# Autodesk Inventor assembly: Curved Assembly
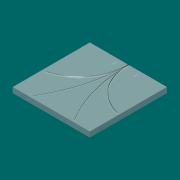
[picture p0: Inventor's stored thumbnail of the model, 180x180]
Saved by Autodesk Inventor 2016 (Build 200138000, 138)
## iProperties
Created: 2015-08-14
Part Number: Curved Assembly
Document SubType Name: Assembly
Designer: Cosmic
Author: Cosmic
## Documents named in this file (4)
- C:\Users\sawaiz\oneDrive\projects\scintillatorPanel\treePanel.iam
- C:\Users\sawaiz\oneDrive\projects\scintillatorPanel\treePanel.ipt
- C:\Users\sawaiz\oneDrive\projects\scintillatorPanel\treeFiberBundle.iam
- C:\Users\sawaiz\oneDrive\projects\scintillatorPanel\Scintillator.xlsx
## Components (2 placed, 2 different names)
1. treePanel:1 — Angle:1, Tangent:2, Flush:1, Mate:27
2. treeFiberBundle:1 [sub-assembly] — Angle:1, Tangent:2, Flush:1, Mate:27
## Relationships (4: Angle 1, Tangent 1, Flush 1, Mate 1)
- Angle:1 (-90 deg): treePanel:1 ↔ treeFiberBundle:1
- Tangent:2 (0.15 mm): treePanel:1 ↔ treeFiberBundle:1
- Flush:1: treePanel:1 ↔ treeFiberBundle:1
- Mate:27: treePanel:1 ↔ treeFiberBundle:1
## Named parameters: OpticalFiberClearence = 0.15 mm, MPPCClearence = 0.075 mm, FiberSensorClerence = 0.5 mm, OpticalFiberDiameter = 1 mm, ScintillatorThickness = 10 mm, SmallTrackDiameter = 175 mm, LargeTrackRatio = 3, ScintillatorEdgeClearence = 3 mm, ScintillatorWidth = 145 mm, ScintillatorHeight = 145 mm, ShallowTrackDepth = 1.3 mm, MPPCSensorClearence = 1.45 mm, MPPCSensorOffsett = 2.105 mm, MPPCWidth = 5.9 mm, MPPCHeight = 6.55 mm, FiberEdgeOffsett = 5 mm, MPPCDepth = 0 mm, LongFiberAngle = 30 deg, ShortFiberAngle = 78 deg, LoopLargeTrackRatio = 1.1, LoopSmallTrackDiameter = 90 mm, MountingScrewOffsett = 20 mm, MountingScrewDepth = 4 mm
